# Autodesk Inventor assembly: ENSAMBLE_V3
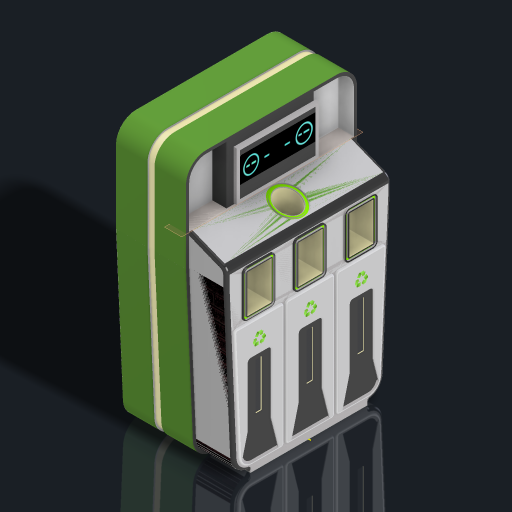
[picture p0: Inventor's stored thumbnail of the model, 512x512]
Saved by Autodesk Inventor 2024.3 (Build 283343000, 343)
## iProperties
Created: 2024-05-12
Part Number: ENSAMBLE_V3
Material: Generic
Document SubType Name: Assembly
Designer: Niler
Author: Niler
## Documents named in this file (10)
- C:\Users\Niler\OneDrive\Escritorio\RECICLADOR\RECICLADOR_MODELO_3D\VERSION_COMPLETA\ENSAMBLE_V3.iam
- C:\Users\Niler\OneDrive\Escritorio\RECICLADOR\RECICLADOR_MODELO_3D\VERSION_COMPLETA\CARCASA_V3.ipt
- C:\Users\Niler\OneDrive\Escritorio\RECICLADOR\RECICLADOR_MODELO_3D\VERSION_COMPLETA\DIMENSIONES_PANTALLA_22.ipt
- C:\Users\Niler\OneDrive\Escritorio\RECICLADOR\RECICLADOR_MODELO_3D\PIEZAS\CARCASA_ALUM_3.ipt
- C:\Users\Niler\OneDrive\Escritorio\RECICLADOR\RECICLADOR_MODELO_3D\PIEZAS\CARCASA_ALUM_4.ipt
- C:\Users\Niler\OneDrive\Escritorio\RECICLADOR\RECICLADOR_MODELO_3D\PIEZAS\CARCASA_ALUM_2.ipt
- C:\Users\Niler\OneDrive\Escritorio\RECICLADOR\RECICLADOR_MODELO_3D\PIEZAS\CARCASA_ALUM_5.ipt
- C:\Users\Niler\OneDrive\Escritorio\RECICLADOR\RECICLADOR_MODELO_3D\PIEZAS\CARCASA_ALUM_6.ipt
- C:\Users\Niler\OneDrive\Escritorio\RECICLADOR\RECICLADOR_MODELO_3D\PIEZAS\CARCASA_ALUM_7.ipt
- C:\Users\Niler\OneDrive\Escritorio\RECICLADOR\RECICLADOR_MODELO_3D\PIEZAS\CARCASA_ALUM_8.ipt
## Components (9 placed, 9 different names)
1. CARCASA_V3:1 — Mate:1, Flush:1, Flush:2, Flush:3, Flush:8, Flush:9, Mate:2, Flush:10, Flush:11, Flush:12, Flush:13, Flush:14, Flush:15, Flush:16, Flush:17, Flush:18, Flush:19, Flush:20, Flush:21
2. DIMENSIONES_PANTALLA_22:1 — Mate:1, Flush:1, Flush:2
3. CARCASA_ALUM_3:1 — Flush:3, Flush:8, Flush:9, Mate:2
4. CARCASA_ALUM_4:1 — Flush:10, Flush:11
5. CARCASA_ALUM_2:1 — Flush:12, Flush:13
6. CARCASA_ALUM_5:1 — Flush:14, Flush:15
7. CARCASA_ALUM_6:1 — Flush:16, Flush:17
8. CARCASA_ALUM_7:1 — Flush:18, Flush:19
9. CARCASA_ALUM_8:1 — Flush:20, Flush:21
## Relationships (19: Flush 17, Mate 2)
- Mate:1: CARCASA_V3:1 ↔ DIMENSIONES_PANTALLA_22:1
- Flush:1 (-16.5 mm): CARCASA_V3:1 ↔ DIMENSIONES_PANTALLA_22:1
- Flush:2 (50 mm): CARCASA_V3:1 ↔ DIMENSIONES_PANTALLA_22:1
- Flush:3: CARCASA_V3:1 ↔ CARCASA_ALUM_3:1
- Flush:8: CARCASA_V3:1 ↔ CARCASA_ALUM_3:1
- Flush:9: CARCASA_V3:1 ↔ CARCASA_ALUM_3:1
- Mate:2: CARCASA_V3:1 ↔ CARCASA_ALUM_3:1
- Flush:10: CARCASA_V3:1 ↔ CARCASA_ALUM_4:1
- Flush:11: CARCASA_V3:1 ↔ CARCASA_ALUM_4:1
- Flush:12: CARCASA_V3:1 ↔ CARCASA_ALUM_2:1
- Flush:13: CARCASA_V3:1 ↔ CARCASA_ALUM_2:1
- Flush:14: CARCASA_V3:1 ↔ CARCASA_ALUM_5:1
- Flush:15: CARCASA_V3:1 ↔ CARCASA_ALUM_5:1
- Flush:16: CARCASA_V3:1 ↔ CARCASA_ALUM_6:1
- Flush:17: CARCASA_V3:1 ↔ CARCASA_ALUM_6:1
- Flush:18: CARCASA_V3:1 ↔ CARCASA_ALUM_7:1
- Flush:19: CARCASA_V3:1 ↔ CARCASA_ALUM_7:1
- Flush:20: CARCASA_V3:1 ↔ CARCASA_ALUM_8:1
- Flush:21: CARCASA_V3:1 ↔ CARCASA_ALUM_8:1
